# Autodesk Inventor assembly: Papa John Test- Ty
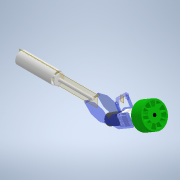
[picture p0: Inventor's stored thumbnail of the model, 180x180]
Saved by Autodesk Inventor 2020 (Build 240168000, 168)
## iProperties
Created: 2020-01-31
Part Number: Papa John Test- Ty
Document SubType Name: Assembly
Designer: aidan
Author: aidan
## Documents named in this file (11)
- C:\Users\aidan\Desktop\T3 Robotics\CAD\Papa John Test- Ty.iam
- C:\Users\aidan\Desktop\T3 Robotics\CAD\Papa John Bolt Plate.ipt
- C:\Users\aidan\Desktop\T3 Robotics\CAD\Generic and Stock\VersaPlanetary Parts\VersaPlanetary Two Stage 775.iam
- C:\Users\aidan\Desktop\T3 Robotics\CAD\Tony's CAD\Compliance wheel.ipt
- C:\Users\aidan\Desktop\T3 Robotics\CAD\Thundershaft 2in.ipt
- C:\Users\aidan\Desktop\T3 Robotics\CAD\Frame Test for Papa John.ipt
- C:\Users\aidan\Desktop\T3 Robotics\CAD\Papa John Mounting Plate with hinge half 1.ipt
- C:\Users\aidan\Desktop\T3 Robotics\CAD\Papa John Mounting Plate with hinge half 2.ipt
- C:\Users\aidan\Desktop\T3 Robotics\CAD\Basic Piston - Outer.ipt
- C:\Users\aidan\Desktop\T3 Robotics\CAD\Basic Piston - Inner.ipt
- C:\Users\aidan\Desktop\T3 Robotics\CAD\Papa John Connecter.ipt
## Components (11 placed, 10 different names)
1. Papa John Bolt Plate:1 — Mate:10, Mate:11, Mate:12, Rotational:1, Mate:14, Tangent:1
2. VersaPlanetary Two Stage 775:1 [sub-assembly] — Mate:7, Mate:8, Flush:9, Flush:10, Mate:9, Insert:1, Insert:2
3. Compliance wheel:1 — Flush:7, Flush:8, Mate:6, Mate:7, Mate:8, Flush:11
4. Compliance wheel:2 — Flush:7, Flush:8, Mate:6
5. Thundershaft 2in:1 — Flush:9, Flush:10, Mate:9, Flush:11
6. Frame Test for Papa John:1 — Mate:10, Mate:11, Mate:12, Mate:13
7. Papa John Mounting Plate with hinge half 1:1 — Rotational:1, Insert:1, Insert:2, Rotational:2
8. Papa John Mounting Plate with hinge half 2:1 — Rotational:2, Insert:3
9. Basic Piston - Outer:1 — Mate:13, Mate:14, Tangent:1, Cylindrical:1, Mate:15
10. Basic Piston - Inner:1 — Cylindrical:1, Mate:15, Cylindrical:2
11. Papa John Connecter:1 — Insert:3, Cylindrical:2
## Relationships (23: Mate 10, Flush 5, Insert 3, RevoluteJoint 2, CylindricalJoint 2, Tangent 1)
- Flush:7: Compliance wheel:1 ↔ Compliance wheel:2
- Flush:8: Compliance wheel:1 ↔ Compliance wheel:2
- Mate:6: Compliance wheel:1 ↔ Compliance wheel:2
- Mate:7: VersaPlanetary Two Stage 775:1 ↔ Compliance wheel:1
- Mate:8: VersaPlanetary Two Stage 775:1 ↔ Compliance wheel:1
- Flush:9: VersaPlanetary Two Stage 775:1 ↔ Thundershaft 2in:1
- Flush:10: VersaPlanetary Two Stage 775:1 ↔ Thundershaft 2in:1
- Mate:9: VersaPlanetary Two Stage 775:1 ↔ Thundershaft 2in:1
- Flush:11: Compliance wheel:1 ↔ Thundershaft 2in:1
- Mate:10: Papa John Bolt Plate:1 ↔ Frame Test for Papa John:1
- Mate:11: Papa John Bolt Plate:1 ↔ Frame Test for Papa John:1
- Mate:12: Papa John Bolt Plate:1 ↔ Frame Test for Papa John:1
- Rotational:1 [RevoluteJoint]: Papa John Bolt Plate:1 ↔ Papa John Mounting Plate with hinge half 1:1
- Insert:1: VersaPlanetary Two Stage 775:1 ↔ Papa John Mounting Plate with hinge half 1:1
- Insert:2: VersaPlanetary Two Stage 775:1 ↔ Papa John Mounting Plate with hinge half 1:1
- Rotational:2 [RevoluteJoint]: Papa John Mounting Plate with hinge half 1:1 ↔ Papa John Mounting Plate with hinge half 2:1
- Mate:13: Frame Test for Papa John:1 ↔ Basic Piston - Outer:1
- Mate:14: Papa John Bolt Plate:1 ↔ Basic Piston - Outer:1
- Tangent:1 (48.0314 mm): Papa John Bolt Plate:1 ↔ Basic Piston - Outer:1
- Cylindrical:1: Basic Piston - Outer:1 ↔ Basic Piston - Inner:1
- Mate:15: Basic Piston - Outer:1 ↔ Basic Piston - Inner:1
- Insert:3: Papa John Mounting Plate with hinge half 2:1 ↔ Papa John Connecter:1
- Cylindrical:2: Basic Piston - Inner:1 ↔ Papa John Connecter:1
